# Autodesk Inventor assembly: Full Assembly
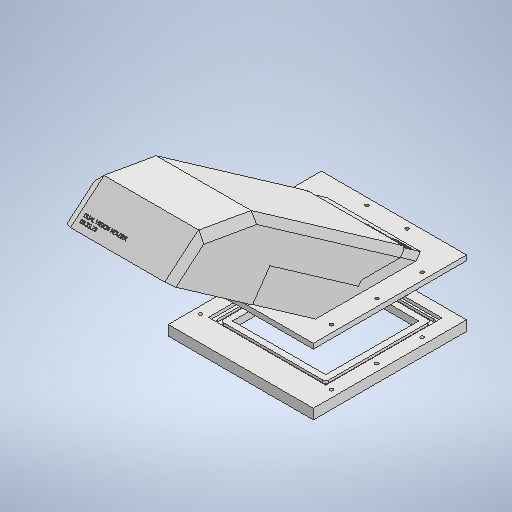
[picture p0: Inventor's stored thumbnail of the model, 512x512]
Saved by Autodesk Inventor 2025.3 (Build 293356030, 356C)
## iProperties
Created: 2025-08-13
Part Number: Full Assembly
Document SubType Name: Assembly
Designer: mateo
Author: mateo
## Documents named in this file (4)
- C:\GitHub\In-situ-monitoring-of-powder-bed-fusion-additive-manufacturing\system_development\Damascus\v0.5\Full Assembly.iam
- C:\GitHub\In-situ-monitoring-of-powder-bed-fusion-additive-manufacturing\system_development\Damascus\v0.5\parts\Glass holder.ipt
- C:\GitHub\In-situ-monitoring-of-powder-bed-fusion-additive-manufacturing\system_development\Damascus\v0.5\parts\cameraholderbody v0.5.ipt
- C:\GitHub\In-situ-monitoring-of-powder-bed-fusion-additive-manufacturing\system_development\Damascus\v0.5\parts\cameraholderlid v0.5.ipt
## Components (3 placed, 3 different names)
1. Glass holder:1 — Insert:1
2. cameraholderbody v0.5:1 — Insert:1, Mate:1, Mate:2
3. cameraholderlid v0.5:1 — Mate:1, Mate:2
## Relationships (3: Mate 2, Insert 1)
- Insert:1 (50.8 mm): Glass holder:1 ↔ cameraholderbody v0.5:1
- Mate:1: cameraholderbody v0.5:1 ↔ cameraholderlid v0.5:1
- Mate:2: cameraholderbody v0.5:1 ↔ cameraholderlid v0.5:1
